# Autodesk Inventor assembly: Escovão
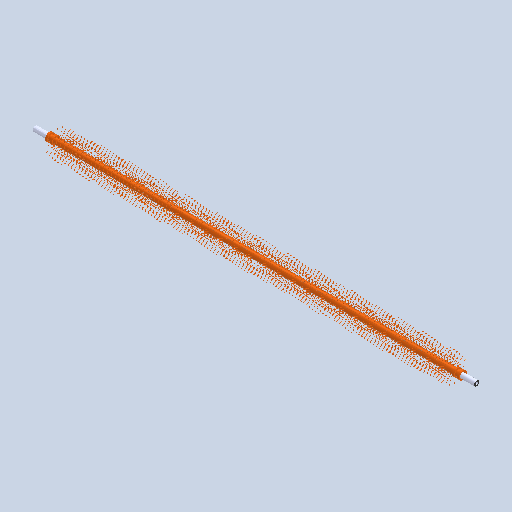
[picture p0: Inventor's stored thumbnail of the model, 512x512]
Saved by Autodesk Inventor 2025.3 (Build 293356030, 356C)
## iProperties
Created: 2026-01-08
Part Number: Escovão
Document SubType Name: Assembly
Designer: Rubens
Author: Rubens
## Documents named in this file (3)
- C:\Users\Rubens\Downloads\Limpador\Escovão.iam
- C:\Users\Rubens\Downloads\Limpador\EscovãoMID.ipt
- C:\Users\Rubens\Downloads\Limpador\EscovãoInicial.ipt
## Components (3 placed, 2 different names)
1. EscovãoMID:1 — Coincidente:2, Coincidente:3
2. EscovãoInicial:1
3. EscovãoInicial:2 — Coincidente:2, Coincidente:3
## Relationships (3: Mate 3)
- [Mate]: EscovãoMID:1 ↔ EscovãoInicial:1
- Coincidente:2 [Mate]: EscovãoMID:1 ↔ EscovãoInicial:2
- Coincidente:3 [Mate]: EscovãoMID:1 ↔ EscovãoInicial:2
